# Autodesk Inventor assembly: frame assembly 3
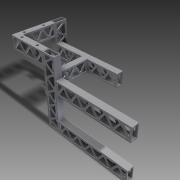
[picture p0: Inventor's stored thumbnail of the model, 180x180]
Saved by Autodesk Inventor 2012 (Build 160160000, 160)
## iProperties
Created: 2013-01-04
Part Number: frame assembly 3
Document SubType Name: Assembly
Designer: Bryce
Author: Bryce
## Documents named in this file (6)
- C:\Users\Bryce\Dropbox\Inventor Design Project Files\Independent Swerves\Inventor 2012\frame assembly 3.iam
- C:\Users\Bryce\Dropbox\Inventor Design Project Files\Independent Swerves\Inventor 2012\right fram piece 3.ipt
- C:\Users\Bryce\Dropbox\Inventor Design Project Files\Independent Swerves\Inventor 2012\vertical frame piece2.ipt
- C:\Users\Bryce\Dropbox\Inventor Design Project Files\Independent Swerves\Inventor 2012\small L bracket.ipt
- C:\Users\Bryce\Dropbox\Inventor Design Project Files\Independent Swerves\Inventor 2012\5in 2by1 frame piece.ipt
- C:\Users\Bryce\Dropbox\Inventor Design Project Files\Independent Swerves\Inventor 2012\left frame piece 3.ipt
## Components (10 placed, 5 different names)
1. left frame piece 3:1 — Mate:1, Mate:2, Flush:1, Mate:4, Flush:4, Flush:5, Mate:17
2. right fram piece 3:1 — Mate:1, Mate:2, Flush:1, Mate:3, Flush:2, Flush:3
3. vertical frame piece2:1 — Mate:3, Flush:2, Flush:3, Mate:5, Flush:6, Mate:7, Flush:10, Flush:11, Mate:10, Flush:18, Mate:19, Flush:22
4. vertical frame piece2:2 — Mate:4, Flush:4, Flush:5, Mate:9, Flush:16, Mate:18, Flush:20
5. vertical frame piece2:4 — Mate:7, Flush:10, Flush:11
6. vertical frame piece2:5 — Mate:5, Flush:6
7. small L bracket:1 — Mate:9, Flush:16, Mate:17, Flush:19
8. small L bracket:2 — Mate:10, Flush:18, Flush:19
9. vertical frame piece2:7 — Mate:18, Flush:20, Flush:23
10. 5in 2by1 frame piece:1 — Mate:19, Flush:22, Flush:23
## Relationships (25: Flush 14, Mate 11)
- Mate:1: left frame piece 3:1 ↔ right fram piece 3:1
- Mate:2: left frame piece 3:1 ↔ right fram piece 3:1
- Flush:1: left frame piece 3:1 ↔ right fram piece 3:1
- Mate:3: right fram piece 3:1 ↔ vertical frame piece2:1
- Flush:2: right fram piece 3:1 ↔ vertical frame piece2:1
- Flush:3: right fram piece 3:1 ↔ vertical frame piece2:1
- Mate:4: left frame piece 3:1 ↔ vertical frame piece2:2
- Flush:4: left frame piece 3:1 ↔ vertical frame piece2:2
- Flush:5: left frame piece 3:1 ↔ vertical frame piece2:2
- Mate:5: vertical frame piece2:1 ↔ vertical frame piece2:5
- Flush:6: vertical frame piece2:1 ↔ vertical frame piece2:5
- Mate:7: vertical frame piece2:1 ↔ vertical frame piece2:4
- Flush:10: vertical frame piece2:1 ↔ vertical frame piece2:4
- Flush:11: vertical frame piece2:1 ↔ vertical frame piece2:4
- Mate:9: vertical frame piece2:2 ↔ small L bracket:1
- Flush:16: vertical frame piece2:2 ↔ small L bracket:1
- Mate:17 (76.2 mm): left frame piece 3:1 ↔ small L bracket:1
- Mate:10: vertical frame piece2:1 ↔ small L bracket:2
- Flush:18: vertical frame piece2:1 ↔ small L bracket:2
- Flush:19: small L bracket:1 ↔ small L bracket:2
- Mate:18: vertical frame piece2:2 ↔ vertical frame piece2:7
- Flush:20: vertical frame piece2:2 ↔ vertical frame piece2:7
- Mate:19: vertical frame piece2:1 ↔ 5in 2by1 frame piece:1
- Flush:22: vertical frame piece2:1 ↔ 5in 2by1 frame piece:1
- Flush:23: vertical frame piece2:7 ↔ 5in 2by1 frame piece:1
